# Autodesk Inventor assembly: Assembly3
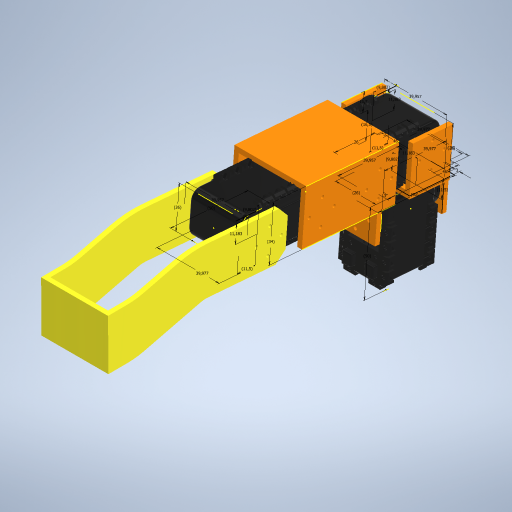
[picture p0: Inventor's stored thumbnail of the model, 512x512]
Saved by Autodesk Inventor 2024 (Build 280153000, 153)
## iProperties
Created: 2024-02-16
Part Number: Assembly3
Document SubType Name: Assembly
Designer: kamil
Author: kamil
## Documents named in this file (6)
- D:\Projects\Robotics\Hexapod\Assembly3.iam
- D:\Projects\Robotics\Hexapod\first_junction.ipt
- D:\Projects\Robotics\Hexapod\AX-12A\AX-12A.iam
- D:\Projects\Robotics\Hexapod\second_junction.ipt
- D:\Projects\Robotics\Hexapod\leg_part.ipt
- D:\Projects\Robotics\Hexapod\AX-12A\ASM0002_ASM.iam
## Components (6 placed, 5 different names)
1. first_junction:1 — Mate:1, Mate:2, Mate:3, Mate:10, Mate:11, Mate:12
2. AX-12A:1 [sub-assembly] — Mate:1, Mate:2, Mate:3, Mate:4, Mate:5, Mate:6
3. second_junction:1 — Mate:4, Mate:5, Mate:6, Mate:13, Mate:14, Mate:15
4. ASM0002_ASM:1 [sub-assembly] — Mate:13, Mate:14, Mate:15, Mate:16, Mate:17, Mate:18
5. ASM0002_ASM:2 [sub-assembly] — Mate:10, Mate:11, Mate:12
6. leg_part:1 — Mate:16, Mate:17, Mate:18
## Relationships (15: Mate 15)
- Mate:1: first_junction:1 ↔ AX-12A:1
- Mate:2: first_junction:1 ↔ AX-12A:1
- Mate:3: first_junction:1 ↔ AX-12A:1
- Mate:4: AX-12A:1 ↔ second_junction:1
- Mate:5: AX-12A:1 ↔ second_junction:1
- Mate:6: AX-12A:1 ↔ second_junction:1
- Mate:10: first_junction:1 ↔ ASM0002_ASM:2
- Mate:11: first_junction:1 ↔ ASM0002_ASM:2
- Mate:12: first_junction:1 ↔ ASM0002_ASM:2
- Mate:13: second_junction:1 ↔ ASM0002_ASM:1
- Mate:14: second_junction:1 ↔ ASM0002_ASM:1
- Mate:15: second_junction:1 ↔ ASM0002_ASM:1
- Mate:16: ASM0002_ASM:1 ↔ leg_part:1
- Mate:17: ASM0002_ASM:1 ↔ leg_part:1
- Mate:18: ASM0002_ASM:1 ↔ leg_part:1
